# Autodesk Inventor assembly: Assembly1
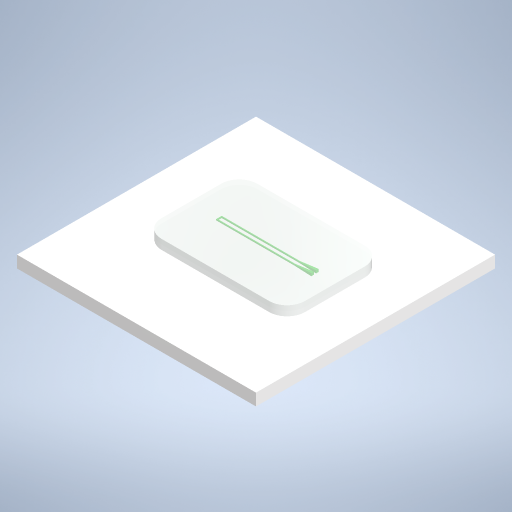
[picture p0: Inventor's stored thumbnail of the model, 512x512]
Saved by Autodesk Inventor 2024.2 (Build 282272000, 272)
## iProperties
Created: 2025-02-11
Part Number: Assembly1
Document SubType Name: Assembly
Designer: Tom
Author: Tom
## Documents named in this file (4)
- C:\Users\Tom\Desktop\UCSF\Preeya UCB\stretchable project\Strain-Sensor-\CAD Files\sensor fab\Assembly1.iam
- C:\Users\Tom\Desktop\UCSF\Preeya UCB\stretchable project\Strain-Sensor-\CAD Files\sensor fab\base plate.ipt
- C:\Users\Tom\Desktop\UCSF\Preeya UCB\stretchable project\Strain-Sensor-\CAD Files\sensor fab\bottom ecoflex layer.ipt
- C:\Users\Tom\Desktop\UCSF\Preeya UCB\stretchable project\Strain-Sensor-\CAD Files\sensor fab\basic strain gauge 0p02.ipt
## Components (4 placed, 3 different names)
1. base plate:1 — Mate:1
2. bottom ecoflex layer:1 — Mate:1, Mate:2, Mate:3, Flush:1, Flush:2
3. basic strain gauge 0p02:1 — Mate:2
4. bottom ecoflex layer:2 — Mate:3, Flush:1, Flush:2
## Relationships (5: Mate 3, Flush 2)
- Mate:1: base plate:1 ↔ bottom ecoflex layer:1
- Mate:2: bottom ecoflex layer:1 ↔ basic strain gauge 0p02:1
- Mate:3: bottom ecoflex layer:1 ↔ bottom ecoflex layer:2
- Flush:1: bottom ecoflex layer:1 ↔ bottom ecoflex layer:2
- Flush:2: bottom ecoflex layer:1 ↔ bottom ecoflex layer:2
